# Autodesk Inventor assembly: stay3
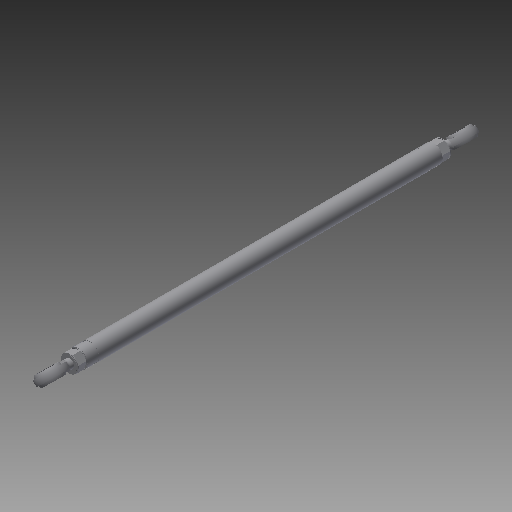
[picture p0: Inventor's stored thumbnail of the model, 512x512]
Saved by Autodesk Inventor 2018.2 (Build 222227000, 227)
## iProperties
Created: 2018-04-27
Part Number: stay3
Material: 一般
Document SubType Name: Assembly
Designer: ku_sk
Author: ku_sk
## Documents named in this file (3)
- C:\Users\ku_sk\Documents\Inventor\Aero\KS-15\Rr.wing\parts\stay\stay3.iam
- C:\Users\ku_sk\Documents\Inventor\Aero\KS-15\Rr.wing\parts\stay\pipe_16mm_200mm.ipt
- C:\Users\ku_sk\Documents\Inventor\Aero\KS-15\Rr.wing\parts\stay\end\stay end.iam
## Components (3 placed, 2 different names)
1. pipe_16mm_200mm:1 — メイト:1, メイト:2, メイト:3, メイト:4, メイト:5, メイト:6, メイト:7
2. stay end:1 [sub-assembly] — メイト:4, メイト:5
3. stay end:2 [sub-assembly] — メイト:6, メイト:7
## Relationships (7: Mate 7)
- メイト:1 [Mate]: pipe_16mm_200mm:1
- メイト:2 [Mate]: pipe_16mm_200mm:1
- メイト:3 [Mate]: pipe_16mm_200mm:1
- メイト:4 [Mate]: pipe_16mm_200mm:1 ↔ stay end:1
- メイト:5 [Mate]: pipe_16mm_200mm:1 ↔ stay end:1
- メイト:6 [Mate]: pipe_16mm_200mm:1 ↔ stay end:2
- メイト:7 [Mate]: pipe_16mm_200mm:1 ↔ stay end:2
